# Autodesk Inventor assembly: Assembly_Cube_Kinematic_Mirror_90_magnetic
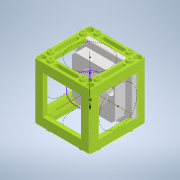
[picture p0: Inventor's stored thumbnail of the model, 180x180]
Saved by Autodesk Inventor 2022 (Build 260153000, 153)
## iProperties
Created: 2022-09-25
Part Number: Assembly_Cube_Kinematic_Mirror_90_magnetic
Document SubType Name: Assembly
Designer: eda_b
Author: eda_b
## Documents named in this file (6)
- G:\My Drive\ASP - M.Sc. Photonics\Practical Modules\MODULE 4 - Master Thesis\2.Experiments\Modules\12.Sample_Mirror_Module\Kinematic_Mirror_Magnetic\Assembly_Cube_Kinematic_Mirror_90_magnetic.iam
- G:\My Drive\ASP - M.Sc. Photonics\Practical Modules\MODULE 4 - Master Thesis\2.Experiments\Modules\2.Base_Cube\Base_Cube_IM\Assembly_Cube_empty_IM_v3.iam
- G:\My Drive\ASP - M.Sc. Photonics\Practical Modules\MODULE 4 - Master Thesis\2.Experiments\Modules\12.Sample_Mirror_Module\Kinematic_Mirror_Magnetic\20_Cube_Insert_Kinematic_45_pro_magnetic_Thorlabs.ipt
- G:\My Drive\ASP - M.Sc. Photonics\Practical Modules\MODULE 4 - Master Thesis\2.Experiments\Modules\12.Sample_Mirror_Module\Kinematic_Mirror_Magnetic\20_Cube_Insert_Kinematic_Mirror_90_pro_magnetic_thin.ipt
- G:\My Drive\ASP - M.Sc. Photonics\Practical Modules\MODULE 4 - Master Thesis\2.Experiments\Modules\12.Sample_Mirror_Module\Kinematic_Mirror_Magnetic\00_NeoDymMagnet_8x3mm.ipt
- G:\My Drive\ASP - M.Sc. Photonics\Practical Modules\MODULE 4 - Master Thesis\2.Experiments\Modules\12.Sample_Mirror_Module\Kinematic_Mirror_Magnetic\00_Thorlabs_PF10-03-P01-Step.ipt
## Components (8 placed, 5 different names)
1. Assembly_Cube_empty_IM_v3:1 [sub-assembly] — Mate:1, Flush:1, Flush:2, Flush:3
2. 20_Cube_Insert_Kinematic_45_pro_magnetic_Thorlabs:1 — Rigid:1, Rotational:3, Rotational:5, Rotational:6
3. 20_Cube_Insert_Kinematic_Mirror_90_pro_magnetic_thin:1 — Mate:1, Flush:1, Flush:2, Flush:3, Rotational:1, Rotational:2, Rigid:1
4. 00_NeoDymMagnet_8x3mm:1 — Rotational:2
5. 00_NeoDymMagnet_8x3mm:2 — Rotational:6
6. 00_NeoDymMagnet_8x3mm:3 — Rotational:5
7. 00_NeoDymMagnet_8x3mm:4 — Rotational:1
8. 00_Thorlabs_PF10-03-P01-Step:1 — Rotational:3
## Relationships (10: RevoluteJoint 5, Flush 3, Mate 1, WeldJoint 1)
- Mate:1: Assembly_Cube_empty_IM_v3:1 ↔ 20_Cube_Insert_Kinematic_Mirror_90_pro_magnetic_thin:1
- Flush:1: Assembly_Cube_empty_IM_v3:1 ↔ 20_Cube_Insert_Kinematic_Mirror_90_pro_magnetic_thin:1
- Flush:2: Assembly_Cube_empty_IM_v3:1 ↔ 20_Cube_Insert_Kinematic_Mirror_90_pro_magnetic_thin:1
- Flush:3: Assembly_Cube_empty_IM_v3:1 ↔ 20_Cube_Insert_Kinematic_Mirror_90_pro_magnetic_thin:1
- Rotational:1 [RevoluteJoint]: 20_Cube_Insert_Kinematic_Mirror_90_pro_magnetic_thin:1 ↔ 00_NeoDymMagnet_8x3mm:4
- Rotational:2 [RevoluteJoint]: 20_Cube_Insert_Kinematic_Mirror_90_pro_magnetic_thin:1 ↔ 00_NeoDymMagnet_8x3mm:1
- Rigid:1 [WeldJoint]: 20_Cube_Insert_Kinematic_45_pro_magnetic_Thorlabs:1 ↔ 20_Cube_Insert_Kinematic_Mirror_90_pro_magnetic_thin:1
- Rotational:3 [RevoluteJoint]: 20_Cube_Insert_Kinematic_45_pro_magnetic_Thorlabs:1 ↔ 00_Thorlabs_PF10-03-P01-Step:1
- Rotational:5 [RevoluteJoint]: 20_Cube_Insert_Kinematic_45_pro_magnetic_Thorlabs:1 ↔ 00_NeoDymMagnet_8x3mm:3
- Rotational:6 [RevoluteJoint]: 20_Cube_Insert_Kinematic_45_pro_magnetic_Thorlabs:1 ↔ 00_NeoDymMagnet_8x3mm:2
